# Autodesk Inventor assembly: parachute_structure_asm
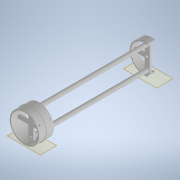
[picture p0: Inventor's stored thumbnail of the model, 180x180]
Saved by Autodesk Inventor 2020 (Build 240168000, 168)
## iProperties
Created: 2022-03-10
Part Number: parachute_structure_asm
Document SubType Name: Assembly
Designer: sp
Author: sp
## Documents named in this file (4)
- C:\Users\sp\Documents\Rocket\rocket\CAD\parachute_structure_asm.iam
- C:\Users\sp\Documents\Rocket\rocket\CAD\stange.ipt
- C:\Users\sp\Documents\Rocket\rocket\CAD\Verbindungsring_2_2.ipt
- C:\Users\sp\Documents\Rocket\rocket\CAD\Verbindungsring_2_3.ipt
## Components (4 placed, 3 different names)
1. stange:1 — Einfügen:1, Einfügen:3
2. stange:2 — Einfügen:2
3. Verbindungsring_2_2:1 — Einfügen:1, Einfügen:2
4. Verbindungsring_2_3:1 — Einfügen:3
## Relationships (3: Insert 3)
- Einfügen:1 [Insert]: stange:1 ↔ Verbindungsring_2_2:1
- Einfügen:2 [Insert]: stange:2 ↔ Verbindungsring_2_2:1
- Einfügen:3 [Insert]: stange:1 ↔ Verbindungsring_2_3:1
